# Autodesk Inventor assembly: Feeder
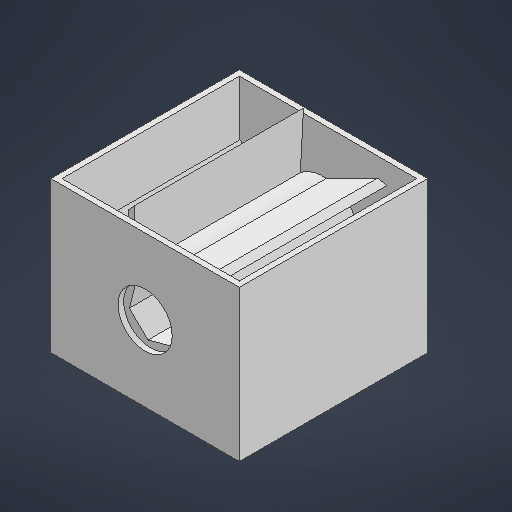
[picture p0: Inventor's stored thumbnail of the model, 512x512]
Saved by Autodesk Inventor 2026.1 (Build 301233000, 233)
## iProperties
Created: 2025-11-03
Part Number: Feeder
Document SubType Name: Assembly
Designer: randy
Author: randy
## Documents named in this file (6)
- C:\Users\uu-112\Documents\Dog Feeder\Feeder.iam
- C:\Users\uu-112\Documents\Dog Feeder\Container.ipt
- C:\Users\uu-112\Documents\Dog Feeder\Spiral.ipt
- C:\Users\uu-112\Documents\Dog Feeder\Shaft.ipt
- C:\Users\uu-112\Documents\Dog Feeder\Spiral 2.ipt
- C:\Users\uu-112\Documents\Dog Feeder\Shaft-EndCap.ipt
## Components (5 placed, 5 different names)
1. Container:1 — Flush:1, Flush:2, Flush:3, Mate:5, Mate:6, Mate:7, Mate:8, Mate:10
2. Spiral:1 — Mate:4, Mate:5, Mate:6
3. Shaft:1 — Mate:4, Mate:7, Mate:8, Mate:9, Mate:11
4. Spiral 2:1 — Mate:9
5. Shaft-EndCap:1 — Mate:10, Mate:11
## Relationships (11: Mate 8, Flush 3)
- Flush:1: Container:1
- Flush:2: Container:1
- Flush:3: Container:1
- Mate:4: Spiral:1 ↔ Shaft:1
- Mate:5: Container:1 ↔ Spiral:1
- Mate:6 (1.27 mm): Container:1 ↔ Spiral:1
- Mate:7: Container:1 ↔ Shaft:1
- Mate:8: Container:1 ↔ Shaft:1
- Mate:9: Shaft:1 ↔ Spiral 2:1
- Mate:10: Container:1 ↔ Shaft-EndCap:1
- Mate:11: Shaft:1 ↔ Shaft-EndCap:1
